# Autodesk Inventor assembly: Rail_Assembly
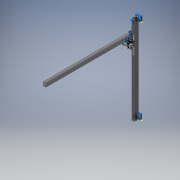
[picture p0: Inventor's stored thumbnail of the model, 180x180]
Saved by Autodesk Inventor 2019.4 (Build 234330000, 330)
## iProperties
Created: 2021-01-26
Part Number: Rail_Assembly
Document SubType Name: Assembly
Designer: Jorian Brusind
Mass: 3786.54 g
Surface Area: 19508.5 cm^2
Volume: 2323.9 cm^3
Density: 1.62939 g/cm^3
Author: Jorian Brusind
## Documents named in this file (17)
- C:\Users\Jorian Brusind\Documents\GitHub\PersonalProjects\HyperRail\Inventor Files\Rail_Assembly.iam
- C:\Users\Jorian Brusind\Documents\GitHub\PersonalProjects\Inventor Projects\Useful models\NEMA_Steppers\NEMA23\23HS8430B.ipt
- C:\Users\Jorian Brusind\Documents\GitHub\PersonalProjects\HyperRail\Inventor Files\NEMA23_StepperonlineMount.ipt
- C:\Users\Jorian Brusind\Documents\GitHub\PersonalProjects\HyperRail\Inventor Files\Roller_Bracket.iam
- C:\Users\Jorian Brusind\Documents\GitHub\PersonalProjects\HyperRail\Inventor Files\LargeBelt_Pulley.ipt
- C:\Users\Jorian Brusind\Documents\GitHub\PersonalProjects\Inventor Projects\Useful models\8020_Sets\IPT_40_Series\Extra_40_Series\HFS5-4060-4000\HFS5-4060-1275.ipt
- C:\Users\Jorian Brusind\Documents\GitHub\PersonalProjects\Inventor Projects\Useful models\8020_Sets\IPT_20_Series\IPT_20_Series\20-2040_200mm.ipt
- C:\Users\Jorian Brusind\Documents\GitHub\PersonalProjects\HyperRail\Inventor Files\2804S_NEMA2115_1Gearbox.ipt
- C:\Users\Jorian Brusind\Documents\GitHub\PersonalProjects\HyperRail\Inventor Files\Large_Belt.ipt
- C:\Users\Jorian Brusind\Documents\GitHub\PersonalProjects\HyperRail\Inventor Files\Belt_Clamp.ipt
- C:\Users\Jorian Brusind\Documents\GitHub\PersonalProjects\Inventor Projects\Useful models\8020_Sets\IPT_40_Series\Extra_40_Series\90deg_4040.ipt
- C:\Users\Jorian Brusind\Documents\GitHub\PersonalProjects\HyperRail\Inventor Files\11mm_BearingWheel.ipt
- C:\Users\Jorian Brusind\Documents\GitHub\PersonalProjects\HyperRail\Inventor Files\63_5mmSpacer.ipt
- C:\Users\Jorian Brusind\Documents\GitHub\PersonalProjects\HyperRail\Inventor Files\Bottom_Stand.ipt
- C:\Users\Jorian Brusind\Documents\GitHub\PersonalProjects\HyperRail\Inventor Files\RightAngle_Bracket.ipt
- C:\Users\Jorian Brusind\Documents\GitHub\PersonalProjects\HyperRail\Inventor Files\Belt_Clamp_R.ipt
- C:\Users\Jorian Brusind\Documents\GitHub\PersonalProjects\Inventor Projects\Useful models\Metric bolt\Bolt M5 50mm.ipt
## Components (22 placed, 16 different names)
1. 23HS8430B:1 — Mate:24, Angle:1, Mate:48, Mate:97
2. NEMA23_StepperonlineMount:1 — Mate:24, Angle:1, Angle:2, Mate:57, Flush:14, Mate:98, Mate:99, Flush:37, Mate:103, Flush:38
3. Roller_Bracket:1 [sub-assembly] — Mate:78, Flush:29, Flush:31, Flush:32, Mate:81, Flush:33
4. Roller_Bracket:2 [sub-assembly] — Mate:79, Flush:30, Mate:80, Flush:31, Flush:32
5. LargeBelt_Pulley:1 — Mate:50, Mate:51, Flush:20, Mate:74, Mate:75
6. HFS5-4060-1275:1 — Flush:20, Mate:70, Flush:22, Mate:71, Mate:72, Flush:23, Mate:73, Flush:24, Flush:25, Flush:26, Mate:80, Mate:81, Mate:91, Mate:92, Mate:93, Mate:94, Mate:95, Mate:96, Mate:104, Flush:39, Flush:40, Mate:105
7. HFS5-4060-1275:2 — Flush:10, Mate:56, Mate:57, Flush:14, Mate:82, Mate:84, Mate:86, Mate:88, Mate:100, Mate:102
8. 20-2040_200mm:1 — Flush:10, Mate:56, Mate:78, Flush:29, Mate:79, Flush:30, Flush:33, Flush:34, Mate:83, Flush:35, Flush:36, Mate:85
9. 2804S_NEMA2115_1Gearbox:1 — Mate:48, Angle:2, Mate:50, Mate:51, Mate:97, Mate:98
10. Large_Belt:1 — Mate:72, Flush:23, Mate:75
11. Large_Belt:2 — Mate:73, Flush:24, Mate:74
12. Belt_Clamp:1 — Flush:25, Flush:26, Mate:104
13. 90deg_4040:1 — Mate:82, Flush:34, Mate:83, Flush:35
14. 90deg_4040:2 — Mate:84, Flush:36, Mate:85
15. 11mm_BearingWheel:1 — Mate:89, Mate:90, Mate:106, Mate:107
16. 63_5mmSpacer:1 — Mate:86, Mate:88, Mate:89, Mate:90, Mate:101
17. Bottom_Stand:1 — Mate:91, Mate:92, Mate:93
18. Bottom_Stand:2 — Mate:94, Mate:95, Mate:96
19. RightAngle_Bracket:1 — Mate:99, Mate:100, Mate:101, Flush:37
20. RightAngle_Bracket:2 — Mate:102, Mate:103, Flush:38
21. Belt_Clamp_R:1 — Flush:39, Flush:40, Mate:105
22. Bolt M5 50mm:1 — Mate:106, Mate:107
## Relationships (63: Mate 41, Flush 20, Angle 2)
- Mate:24: 23HS8430B:1 ↔ NEMA23_StepperonlineMount:1
- Angle:1 (0 deg): 23HS8430B:1 ↔ NEMA23_StepperonlineMount:1
- Flush:10: HFS5-4060-1275:2 ↔ 20-2040_200mm:1
- Mate:48: 23HS8430B:1 ↔ 2804S_NEMA2115_1Gearbox:1
- Angle:2 (0 deg): NEMA23_StepperonlineMount:1 ↔ 2804S_NEMA2115_1Gearbox:1
- Mate:50: LargeBelt_Pulley:1 ↔ 2804S_NEMA2115_1Gearbox:1
- Mate:51 (3 mm): LargeBelt_Pulley:1 ↔ 2804S_NEMA2115_1Gearbox:1
- Mate:56: HFS5-4060-1275:2 ↔ 20-2040_200mm:1
- Mate:57: NEMA23_StepperonlineMount:1 ↔ HFS5-4060-1275:2
- Flush:14 (-60 mm): NEMA23_StepperonlineMount:1 ↔ HFS5-4060-1275:2
- Flush:20: LargeBelt_Pulley:1 ↔ HFS5-4060-1275:1
- Mate:70: HFS5-4060-1275:1
- Flush:22: HFS5-4060-1275:1
- Mate:71: HFS5-4060-1275:1
- Mate:72: HFS5-4060-1275:1 ↔ Large_Belt:1
- Flush:23 (2.5 mm): HFS5-4060-1275:1 ↔ Large_Belt:1
- Mate:73: HFS5-4060-1275:1 ↔ Large_Belt:2
- Flush:24 (2.5 mm): HFS5-4060-1275:1 ↔ Large_Belt:2
- Mate:74 (25 mm): LargeBelt_Pulley:1 ↔ Large_Belt:2
- Mate:75 (25 mm): LargeBelt_Pulley:1 ↔ Large_Belt:1
- Flush:25 (-2.5 mm): HFS5-4060-1275:1 ↔ Belt_Clamp:1
- Flush:26: HFS5-4060-1275:1 ↔ Belt_Clamp:1
- Mate:78: Roller_Bracket:1 ↔ 20-2040_200mm:1
- Flush:29: Roller_Bracket:1 ↔ 20-2040_200mm:1
- Mate:79: Roller_Bracket:2 ↔ 20-2040_200mm:1
- Flush:30: Roller_Bracket:2 ↔ 20-2040_200mm:1
- Mate:80 (2 mm): Roller_Bracket:2 ↔ HFS5-4060-1275:1
- Flush:31 (2 mm): Roller_Bracket:1 ↔ Roller_Bracket:2
- Flush:32: Roller_Bracket:1 ↔ Roller_Bracket:2
- Mate:81 (2.5 mm): Roller_Bracket:1 ↔ HFS5-4060-1275:1
- Flush:33 (44.5 mm): Roller_Bracket:1 ↔ 20-2040_200mm:1
- Mate:82: HFS5-4060-1275:2 ↔ 90deg_4040:1
- Flush:34: 20-2040_200mm:1 ↔ 90deg_4040:1
- Mate:83: 20-2040_200mm:1 ↔ 90deg_4040:1
- Flush:35: 20-2040_200mm:1 ↔ 90deg_4040:1
- Mate:84: HFS5-4060-1275:2 ↔ 90deg_4040:2
- Flush:36: 20-2040_200mm:1 ↔ 90deg_4040:2
- Mate:85: 20-2040_200mm:1 ↔ 90deg_4040:2
- Mate:86: HFS5-4060-1275:2 ↔ 63_5mmSpacer:1
- Mate:88 (3 mm): HFS5-4060-1275:2 ↔ 63_5mmSpacer:1
- Mate:89: 11mm_BearingWheel:1 ↔ 63_5mmSpacer:1
- Mate:90: 11mm_BearingWheel:1 ↔ 63_5mmSpacer:1
- Mate:91: HFS5-4060-1275:1 ↔ Bottom_Stand:1
- Mate:92: HFS5-4060-1275:1 ↔ Bottom_Stand:1
- Mate:93: HFS5-4060-1275:1 ↔ Bottom_Stand:1
- Mate:94: HFS5-4060-1275:1 ↔ Bottom_Stand:2
- Mate:95: HFS5-4060-1275:1 ↔ Bottom_Stand:2
- Mate:96: HFS5-4060-1275:1 ↔ Bottom_Stand:2
- Mate:97: 23HS8430B:1 ↔ 2804S_NEMA2115_1Gearbox:1
- Mate:98: NEMA23_StepperonlineMount:1 ↔ 2804S_NEMA2115_1Gearbox:1
- Mate:99: NEMA23_StepperonlineMount:1 ↔ RightAngle_Bracket:1
- Mate:100: HFS5-4060-1275:2 ↔ RightAngle_Bracket:1
- Mate:101: 63_5mmSpacer:1 ↔ RightAngle_Bracket:1
- Flush:37 (0.6 mm): NEMA23_StepperonlineMount:1 ↔ RightAngle_Bracket:1
- Mate:102: HFS5-4060-1275:2 ↔ RightAngle_Bracket:2
- Mate:103: NEMA23_StepperonlineMount:1 ↔ RightAngle_Bracket:2
- Flush:38 (0.6 mm): NEMA23_StepperonlineMount:1 ↔ RightAngle_Bracket:2
- Mate:104: HFS5-4060-1275:1 ↔ Belt_Clamp:1
- Flush:39: HFS5-4060-1275:1 ↔ Belt_Clamp_R:1
- Flush:40 (-2.5 mm): HFS5-4060-1275:1 ↔ Belt_Clamp_R:1
- Mate:105: HFS5-4060-1275:1 ↔ Belt_Clamp_R:1
- Mate:106: 11mm_BearingWheel:1 ↔ Bolt M5 50mm:1
- Mate:107: 11mm_BearingWheel:1 ↔ Bolt M5 50mm:1
